# Autodesk Inventor assembly: GearSet 1
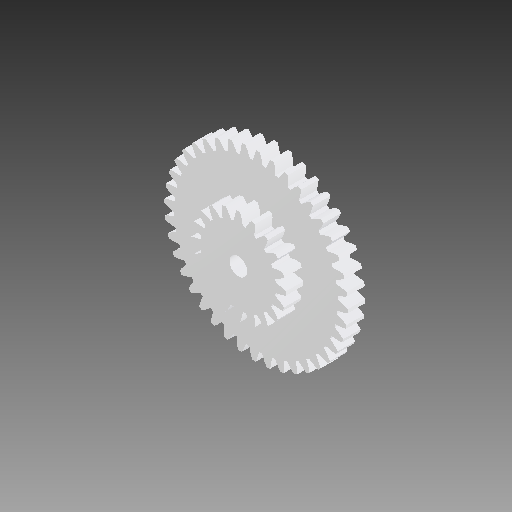
[picture p0: Inventor's stored thumbnail of the model, 512x512]
Saved by Autodesk Inventor 2017 SP1 (Build 210196100, 196)
## iProperties
Created: 2017-09-23
Part Number: GearSet 1
Document SubType Name: Assembly
Designer: Zach
Author: Zach
## Documents named in this file (3)
- C:\Users\Zach\Documents\GitHub\tr1\lib\Gearbox 128;1\GearSet 1.iam
- C:\Users\Zach\Documents\GitHub\tr1\lib\Gearbox 128;1\GearSet 1\Design Accelerator\Spur Gears1.iam
- C:\Users\Zach\Documents\GitHub\tr1\lib\Gearbox 128;1\GearSet 1\Design Accelerator\Spur Gears2.iam
## Components (2 placed, 1 different names)
1. Spur Gears:1 [sub-assembly] — Mate:1, Mate:2
2. Spur Gears:2 [sub-assembly] — Mate:1, Mate:2
## Relationships (2: Mate 2)
- Mate:1: Spur Gears:1 ↔ Spur Gears:2
- Mate:2: Spur Gears:1 ↔ Spur Gears:2
